# Autodesk Inventor assembly: 300-009 (TURNBUCKLE ASSEMBLY)_MIR
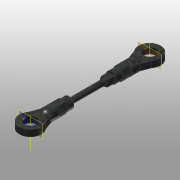
[picture p0: Inventor's stored thumbnail of the model, 180x180]
Saved by Autodesk Inventor 2015 (Build 190159000, 159)
## iProperties
Created: 2015-04-18
Part Number: 300-009 (TURNBUCKLE ASSEMBLY)_MIR
Document SubType Name: Assembly
Designer: Station9
Author: Station9
## Documents named in this file (3)
- D:\Project Archive\AD\AD-6(94.01.29)WSC2011\300-009 (TURNBUCKLE ASSEMBLY)_MIR.iam
- D:\Project Archive\AD\AD-6(94.01.29)WSC2011\500-001_MIR.ipt
- D:\Project Archive\AD\AD-6(94.01.29)WSC2011\500-000_MIR.ipt
## Components (3 placed, 2 different names)
1. 500-001_MIR:1 — Insert:1, Insert:2
2. 500-000_MIR:1 — Insert:1
3. 500-000_MIR:2 — Insert:2
## Relationships (2: Insert 2)
- Insert:1: 500-001_MIR:1 ↔ 500-000_MIR:1
- Insert:2 (-6 mm): 500-001_MIR:1 ↔ 500-000_MIR:2
